# Autodesk Inventor assembly: 5A.00.04.01-IB-VTP-Body-Master-Assy
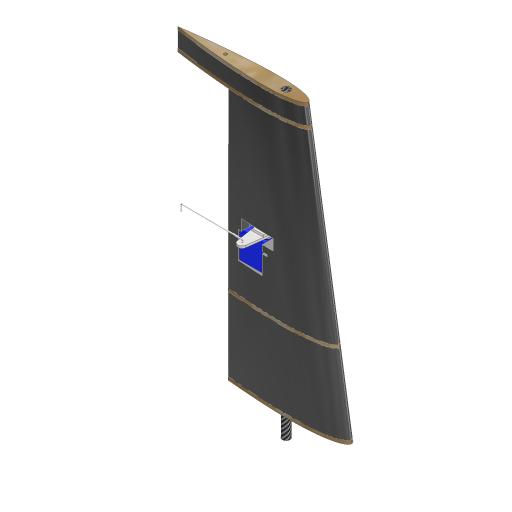
[picture p0: Inventor's stored thumbnail of the model, 512x512]
Saved by Autodesk Inventor 2024.3 (Build 283343000, 343)
## iProperties
Created: 2025-01-14
Part Number: 5A.00.04.01-IB-VTP-Body-Master-Assy
Document SubType Name: Assembly
Designer: inigo
Author: inigo
## Documents named in this file (17)
- C:\Users\inigo\OneDrive - University of Bristol\General - grp-Company A - AVDASI2 2024-25\CAD Files\VTP\5A.00.04.01-IB-VTP-Body-Master-Assy.iam
- C:\Users\inigo\OneDrive - University of Bristol\General - grp-Company A - AVDASI2 2024-25\CAD Files\VTP\5P.00.06.01-IB-VTP-Main-Spar.ipt
- C:\Users\inigo\OneDrive - University of Bristol\General - grp-Company A - AVDASI2 2024-25\CAD Files\VTP\EMAX-09-MD Servo.ipt
- C:\Users\inigo\OneDrive - University of Bristol\General - grp-Company A - AVDASI2 2024-25\CAD Files\VTP\5P.00.02.01-IB-VTP-Body-Final-Right-Second-Rib.ipt
- C:\Users\inigo\OneDrive - University of Bristol\General - grp-Company A - AVDASI2 2024-25\CAD Files\VTP\5P.00.24.01-IB-VTP-Body-Final-Right-Top.ipt
- C:\Users\inigo\OneDrive - University of Bristol\General - grp-Company A - AVDASI2 2024-25\CAD Files\VTP\5P.00.10.01-IB-VTP-Body-Final-Right-Main.ipt
- C:\Users\inigo\OneDrive - University of Bristol\General - grp-Company A - AVDASI2 2024-25\CAD Files\VTP\5P.00.09.01-IB-VTP-Body-Final-Right-Bottom.ipt
- C:\Users\inigo\OneDrive - University of Bristol\General - grp-Company A - AVDASI2 2024-25\CAD Files\VTP\5P.00.11.01-IB-VTP-Body-Final-Top-Rib.ipt
- C:\Users\inigo\OneDrive - University of Bristol\General - grp-Company A - AVDASI2 2024-25\CAD Files\VTP\5P.00.12.01-IB-VTP-Body-Final-Middle-Rib.ipt
- C:\Users\inigo\OneDrive - University of Bristol\General - grp-Company A - AVDASI2 2024-25\CAD Files\VTP\5P.00.13.01-IB-VTP-Body-Final-Bottom-Rib.ipt
- C:\Users\inigo\OneDrive - University of Bristol\General - grp-Company A - AVDASI2 2024-25\CAD Files\VTP\5P.00.14.01-IB-VTP-Body-Final-Left-Top.ipt
- C:\Users\inigo\OneDrive - University of Bristol\General - grp-Company A - AVDASI2 2024-25\CAD Files\VTP\5P.00.15.01-IB-VTP-Body-Final-Left-Bottom.ipt
- C:\Users\inigo\OneDrive - University of Bristol\General - grp-Company A - AVDASI2 2024-25\CAD Files\VTP\5P.00.16.01-IB-VTP-Body-Final-Left-Main.ipt
- C:\Users\inigo\OneDrive - University of Bristol\General - grp-Company A - AVDASI2 2024-25\CAD Files\VTP\5P.00.19.01-IB-VTP-Servo-Horn.ipt
- C:\Users\inigo\OneDrive - University of Bristol\General - grp-Company A - AVDASI2 2024-25\CAD Files\VTP\5P.00.20.01-IB-VTP-Control-Rod.ipt
- C:\Users\inigo\OneDrive - University of Bristol\General - grp-Company A - AVDASI2 2024-25\CAD Files\VTP\5P.00.23.01-IB-VTP-Servo-Rear-Retaining-Rod.ipt
- C:\Users\inigo\OneDrive - University of Bristol\General - grp-Company A - AVDASI2 2024-25\CAD Files\VTP\5P.00.22.01-IB-VTP-Servo-Front-Retaining-Rod.ipt
## Components (16 placed, 16 different names)
1. 5P.00.06.01-IB-VTP-Main-Spar:1 — Mate:1, Flush:1, Mate:3, Mate:6, Mate:9, Mate:12, Mate:14, Mate:16, Mate:18, Mate:20, Mate:29, Mate:51
2. EMAX-09-MD Servo:1 — Mate:22, Mate:23, Mate:24, Mate:25, Mate:27, Mate:48, Mate:49
3. 5P.00.02.01-IB-VTP-Body-Final-Second-Rib:1 — Mate:9, Mate:54, Mate:55, Mate:56
4. 5P.00.24.01-IB-VTP-Body-Final-Right-Top:1 — Mate:6, Mate:57, Mate:75, Mate:77
5. 5P.00.09.01-IB-VTP-Body-Final-Right-Bottom:1 — Mate:20, Mate:21, Mate:52
6. 5P.00.11.01-IB-VTP-Body-Final-Top-Rib:1 — Mate:1, Flush:1, Mate:74, Mate:75, Mate:76, Mate:77
7. 5P.00.12.01-IB-VTP-Body-Final-Middle-Rib:1 — Mate:14, Flush:3, Mate:15, Mate:17, Mate:21
8. 5P.00.13.01-IB-VTP-Body-Final-Bottom-Rib:1 — Mate:18, Mate:19, Flush:5
9. 5P.00.14.01-IB-VTP-Body-Final-Left-Top:1 — Mate:3, Mate:54, Angle:1, Mate:74, Mate:76
10. 5P.00.15.01-IB-VTP-Body-Final-Left-Bottom:1 — Mate:16, Flush:4, Mate:17, Mate:19, Flush:5, Mate:52
11. 5P.00.10.01-IB-VTP-Body-Final-Right-Main:1 — Mate:29, Flush:6, Mate:55
12. 5P.00.16.01-IB-VTP-Body-Final-Left-Main:1 — Mate:12, Flush:3, Mate:15, Flush:4, Mate:22, Mate:23, Mate:24, Mate:26, Mate:28, Flush:6, Mate:56, Angle:1
13. 5P.00.20.01-IB-VTP-Control-Rod:1 — Mate:50
14. 5P.00.23.01-IB-VTP-Servo-Rear-Retaining-Rod:1 — Mate:25, Mate:26
15. 5P.00.22.01-IB-VTP-Servo-Front-Retaining-Rod:1 — Mate:27, Mate:28
16. 5P.00.19.01-IB-VTP-Servo-Horn:1 — Mate:48, Mate:49, Mate:50
## Relationships (40: Mate 34, Flush 5, Angle 1)
- Mate:1: 5P.00.06.01-IB-VTP-Main-Spar:1 ↔ 5P.00.11.01-IB-VTP-Body-Final-Top-Rib:1
- Flush:1: 5P.00.06.01-IB-VTP-Main-Spar:1 ↔ 5P.00.11.01-IB-VTP-Body-Final-Top-Rib:1
- Mate:3: 5P.00.06.01-IB-VTP-Main-Spar:1 ↔ 5P.00.14.01-IB-VTP-Body-Final-Left-Top:1
- Mate:6: 5P.00.06.01-IB-VTP-Main-Spar:1 ↔ 5P.00.24.01-IB-VTP-Body-Final-Right-Top:1
- Mate:9: 5P.00.06.01-IB-VTP-Main-Spar:1 ↔ 5P.00.02.01-IB-VTP-Body-Final-Second-Rib:1
- Mate:12: 5P.00.06.01-IB-VTP-Main-Spar:1 ↔ 5P.00.16.01-IB-VTP-Body-Final-Left-Main:1
- Mate:14: 5P.00.06.01-IB-VTP-Main-Spar:1 ↔ 5P.00.12.01-IB-VTP-Body-Final-Middle-Rib:1
- Flush:3: 5P.00.12.01-IB-VTP-Body-Final-Middle-Rib:1 ↔ 5P.00.16.01-IB-VTP-Body-Final-Left-Main:1
- Mate:15: 5P.00.12.01-IB-VTP-Body-Final-Middle-Rib:1 ↔ 5P.00.16.01-IB-VTP-Body-Final-Left-Main:1
- Mate:16: 5P.00.06.01-IB-VTP-Main-Spar:1 ↔ 5P.00.15.01-IB-VTP-Body-Final-Left-Bottom:1
- Flush:4: 5P.00.15.01-IB-VTP-Body-Final-Left-Bottom:1 ↔ 5P.00.16.01-IB-VTP-Body-Final-Left-Main:1
- Mate:17: 5P.00.12.01-IB-VTP-Body-Final-Middle-Rib:1 ↔ 5P.00.15.01-IB-VTP-Body-Final-Left-Bottom:1
- Mate:18: 5P.00.06.01-IB-VTP-Main-Spar:1 ↔ 5P.00.13.01-IB-VTP-Body-Final-Bottom-Rib:1
- Mate:19: 5P.00.13.01-IB-VTP-Body-Final-Bottom-Rib:1 ↔ 5P.00.15.01-IB-VTP-Body-Final-Left-Bottom:1
- Flush:5: 5P.00.13.01-IB-VTP-Body-Final-Bottom-Rib:1 ↔ 5P.00.15.01-IB-VTP-Body-Final-Left-Bottom:1
- Mate:20: 5P.00.06.01-IB-VTP-Main-Spar:1 ↔ 5P.00.09.01-IB-VTP-Body-Final-Right-Bottom:1
- Mate:21: 5P.00.09.01-IB-VTP-Body-Final-Right-Bottom:1 ↔ 5P.00.12.01-IB-VTP-Body-Final-Middle-Rib:1
- Mate:22: EMAX-09-MD Servo:1 ↔ 5P.00.16.01-IB-VTP-Body-Final-Left-Main:1
- Mate:23: EMAX-09-MD Servo:1 ↔ 5P.00.16.01-IB-VTP-Body-Final-Left-Main:1
- Mate:24: EMAX-09-MD Servo:1 ↔ 5P.00.16.01-IB-VTP-Body-Final-Left-Main:1
- Mate:25: EMAX-09-MD Servo:1 ↔ 5P.00.23.01-IB-VTP-Servo-Rear-Retaining-Rod:1
- Mate:26: 5P.00.16.01-IB-VTP-Body-Final-Left-Main:1 ↔ 5P.00.23.01-IB-VTP-Servo-Rear-Retaining-Rod:1
- Mate:27: EMAX-09-MD Servo:1 ↔ 5P.00.22.01-IB-VTP-Servo-Front-Retaining-Rod:1
- Mate:28: 5P.00.16.01-IB-VTP-Body-Final-Left-Main:1 ↔ 5P.00.22.01-IB-VTP-Servo-Front-Retaining-Rod:1
- Mate:29: 5P.00.06.01-IB-VTP-Main-Spar:1 ↔ 5P.00.10.01-IB-VTP-Body-Final-Right-Main:1
- Flush:6: 5P.00.10.01-IB-VTP-Body-Final-Right-Main:1 ↔ 5P.00.16.01-IB-VTP-Body-Final-Left-Main:1
- Mate:48: EMAX-09-MD Servo:1 ↔ 5P.00.19.01-IB-VTP-Servo-Horn:1
- Mate:49: EMAX-09-MD Servo:1 ↔ 5P.00.19.01-IB-VTP-Servo-Horn:1
- Mate:50: 5P.00.20.01-IB-VTP-Control-Rod:1 ↔ 5P.00.19.01-IB-VTP-Servo-Horn:1
- Mate:51: 5P.00.06.01-IB-VTP-Main-Spar:1
- Mate:52: 5P.00.09.01-IB-VTP-Body-Final-Right-Bottom:1 ↔ 5P.00.15.01-IB-VTP-Body-Final-Left-Bottom:1
- Mate:54: 5P.00.02.01-IB-VTP-Body-Final-Second-Rib:1 ↔ 5P.00.14.01-IB-VTP-Body-Final-Left-Top:1
- Mate:55: 5P.00.02.01-IB-VTP-Body-Final-Second-Rib:1 ↔ 5P.00.10.01-IB-VTP-Body-Final-Right-Main:1
- Mate:56: 5P.00.02.01-IB-VTP-Body-Final-Second-Rib:1 ↔ 5P.00.16.01-IB-VTP-Body-Final-Left-Main:1
- Angle:1 (90 deg): 5P.00.14.01-IB-VTP-Body-Final-Left-Top:1 ↔ 5P.00.16.01-IB-VTP-Body-Final-Left-Main:1
- Mate:57: 5P.00.24.01-IB-VTP-Body-Final-Right-Top:1
- Mate:74: 5P.00.11.01-IB-VTP-Body-Final-Top-Rib:1 ↔ 5P.00.14.01-IB-VTP-Body-Final-Left-Top:1
- Mate:75: 5P.00.24.01-IB-VTP-Body-Final-Right-Top:1 ↔ 5P.00.11.01-IB-VTP-Body-Final-Top-Rib:1
- Mate:76: 5P.00.11.01-IB-VTP-Body-Final-Top-Rib:1 ↔ 5P.00.14.01-IB-VTP-Body-Final-Left-Top:1
- Mate:77: 5P.00.24.01-IB-VTP-Body-Final-Right-Top:1 ↔ 5P.00.11.01-IB-VTP-Body-Final-Top-Rib:1
